# Autodesk Inventor assembly: WormAndMotorizedRingFor3dPrinting
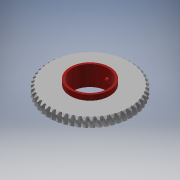
[picture p0: Inventor's stored thumbnail of the model, 180x180]
Saved by Autodesk Inventor 2019.3 (Build 233278000, 278)
## iProperties
Created: 2019-01-22
Part Number: WormAndMotorizedRingFor3dPrinting
Document SubType Name: Assembly
Designer: steele
Author: steele
## Documents named in this file (3)
- C:\git\CAD-Development\robSteele\ShapeWays\TelescopeProjects\Focuser\WormAndMotorizedRingFor3dPrinting.iam
- C:\git\CAD-Development\robSteele\ShapeWays\TelescopeProjects\Focuser\ExternalMotorizedOuterRing.ipt
- C:\git\CAD-Development\robSteele\ShapeWays\TelescopeProjects\Focuser\WormGear1UsedFor3dPrinting.ipt
## Components (2 placed, 2 different names)
1. ExternalMotorizedOuterRing:1 — Insert:1
2. Worm Gear:1 — Insert:1
## Relationships (1: Insert 1)
- Insert:1 (-6.5532 mm): ExternalMotorizedOuterRing:1 ↔ Worm Gear:1
